# Autodesk Inventor assembly: A_U_Boot
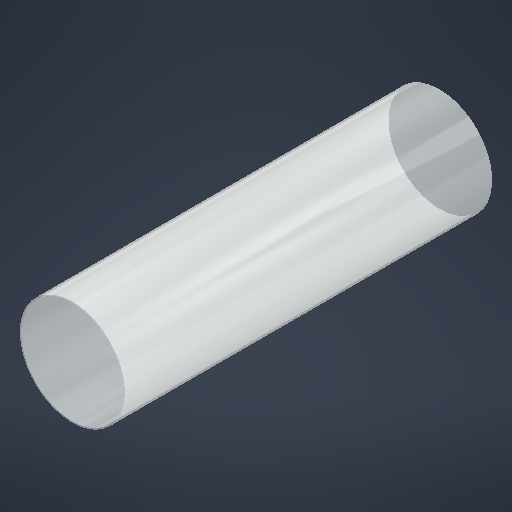
[picture p0: Inventor's stored thumbnail of the model, 512x512]
Saved by Autodesk Inventor 2026 (Build 300175000, 175)
## iProperties
Created: 2025-04-26
Part Number: A_U_Boot
Document SubType Name: Assembly
Designer: FAL
Author: FAL
## Documents named in this file (2)
- C:\Users\FAL\Desktop\git\U-BERT\CAD\A_U-Boot\A_U_Boot.iam
- C:\Users\FAL\Desktop\git\U-BERT\CAD\Trockenzelle\A_Trockenzelle.iam
## Components (1 placed, 1 different names)
1. A_Trockenzelle:1 [sub-assembly] — Fluchtend:1, Passend:1, Passend:2
## Relationships (3: Mate 2, Flush 1)
- Fluchtend:1 [Flush]: A_Trockenzelle:1
- Passend:1 [Mate]: A_Trockenzelle:1
- Passend:2 [Mate]: A_Trockenzelle:1
